# Autodesk Inventor assembly: RollerSmallNoSpacer
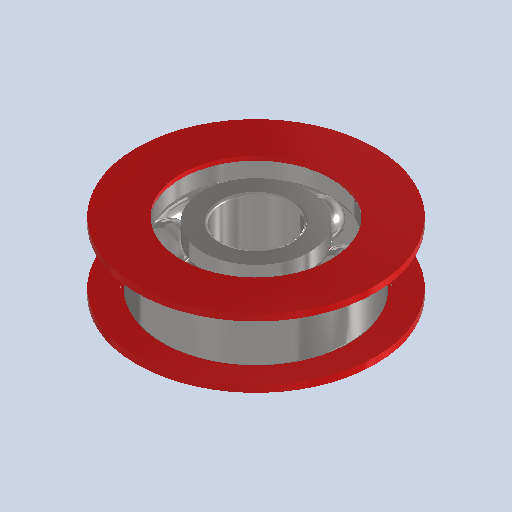
[picture p0: Inventor's stored thumbnail of the model, 512x512]
Saved by Autodesk Inventor 2023 (Build 270158000, 158)
## iProperties
Created: 2023-08-18
Part Number: RollerSmallNoSpacer
Document SubType Name: Assembly
Designer: Felix
Author: Felix
## Documents named in this file (3)
- D:\Programmieren\PineapplePenPlotter\Inventor\try_3\RollerSmallNoSpacer.iam
- C:\Users\Felix\Documents\Inventor\Content Center Files\R2023\en-US\BS 290 SKF(30)\BS 290 SKF - SKF 608.ipt
- D:\Programmieren\PineapplePenPlotter\Inventor\BearingRim.ipt
## Components (3 placed, 2 different names)
1. BS 290 SKF 608:1 — Mate:1, Mate:2, Mate:3, Mate:4
2. BearingRim:1 — Mate:2, Mate:3
3. BearingRim:2 — Mate:1, Mate:4
## Relationships (4: Mate 4)
- Mate:1: BS 290 SKF 608:1 ↔ BearingRim:2
- Mate:2: BS 290 SKF 608:1 ↔ BearingRim:1
- Mate:3: BS 290 SKF 608:1 ↔ BearingRim:1
- Mate:4: BS 290 SKF 608:1 ↔ BearingRim:2
